# Autodesk Inventor assembly: Assembly
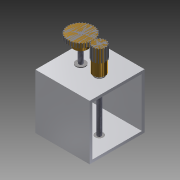
[picture p0: Inventor's stored thumbnail of the model, 180x180]
Saved by Autodesk Inventor 2015 (Build 190159000, 159)
## iProperties
Created: 2015-06-23
Part Number: Assembly
Document SubType Name: Assembly
Designer: kenta
Author: kenta
## Documents named in this file (9)
- C:\Users\kenta\Documents\Inventor\知能ロボコン\Poster presentation\Assembly1.iam
- C:\Users\kenta\Documents\Inventor\知能ロボコン\Poster presentation\Square pipe.ipt
- C:\Users\kenta\Documents\Inventor\知能ロボコン\Poster presentation\Bearing_MF63ZZ.ipt
- C:\Users\kenta\Documents\Inventor\知能ロボコン\Poster presentation\S50B 18K+0803.ipt
- C:\Users\kenta\Documents\Inventor\知能ロボコン\Poster presentation\S50B 36B+0303.ipt
- C:\Users\kenta\Documents\Inventor\知能ロボコン\Poster presentation\Stopper.ipt
- C:\Users\kenta\Documents\Inventor\知能ロボコン\Poster presentation\Shaft 65mm.ipt
- C:\Users\健太\Documents\Inventor\知能ロボコン\Poster presentation\Assembly1\デザイン アクセラレータ\平歯車1.iam
- C:\Users\kenta\Documents\Inventor\知能ロボコン\Poster presentation\Assembly1\デザイン アクセラレータ\平歯車1.iam
## Components (13 placed, 7 different names)
1. Square pipe:1 — 挿入:1, 挿入:2, 挿入:3, 挿入:4, メイト:1
2. Bearing_MF63ZZ:1 — 挿入:1, 挿入:7
3. Bearing_MF63ZZ:2 — 挿入:2, 挿入:8
4. Bearing_MF63ZZ:3 — 挿入:3, 挿入:9
5. Bearing_MF63ZZ:4 — 挿入:4, 挿入:11
6. S50B 18K+0803:1 — 挿入:7, メイト:3, フラッシュ:2, フラッシュ:4
7. S50B 36B+0303:1 — 挿入:8, メイト:2, フラッシュ:1, 挿入:12, メイト:4, フラッシュ:3
8. Stopper:1 — 挿入:11
9. Stopper:2 — 挿入:9, 挿入:10
10. Shaft 65mm:1 — 挿入:10, メイト:5
11. 平歯車:1 [sub-assembly] — メイト:2, フラッシュ:1, メイト:3, フラッシュ:2
12. Shaft 65mm:2 — 挿入:12
13. 平歯車:1 [sub-assembly] — メイト:4, フラッシュ:3, メイト:5, フラッシュ:4
## Relationships (19: Insert 10, Mate 5, Flush 4)
- 挿入:1 [Insert]: Square pipe:1 ↔ Bearing_MF63ZZ:1
- 挿入:2 [Insert]: Square pipe:1 ↔ Bearing_MF63ZZ:2
- 挿入:3 [Insert]: Square pipe:1 ↔ Bearing_MF63ZZ:3
- 挿入:4 [Insert]: Square pipe:1 ↔ Bearing_MF63ZZ:4
- 挿入:7 [Insert] (1 mm): Bearing_MF63ZZ:1 ↔ S50B 18K+0803:1
- 挿入:8 [Insert] (-19 mm): Bearing_MF63ZZ:2 ↔ S50B 36B+0303:1
- 挿入:9 [Insert]: Bearing_MF63ZZ:3 ↔ Stopper:2
- 挿入:10 [Insert]: Stopper:2 ↔ Shaft 65mm:1
- 挿入:11 [Insert]: Bearing_MF63ZZ:4 ↔ Stopper:1
- メイト:1 [Mate]: Square pipe:1
- メイト:2 [Mate]: S50B 36B+0303:1 ↔ 平歯車:1
- フラッシュ:1 [Flush]: S50B 36B+0303:1 ↔ 平歯車:1
- メイト:3 [Mate]: S50B 18K+0803:1 ↔ 平歯車:1
- フラッシュ:2 [Flush]: S50B 18K+0803:1 ↔ 平歯車:1
- 挿入:12 [Insert]: S50B 36B+0303:1 ↔ Shaft 65mm:2
- メイト:4 [Mate]: S50B 36B+0303:1 ↔ 平歯車:1
- フラッシュ:3 [Flush]: S50B 36B+0303:1 ↔ 平歯車:1
- メイト:5 [Mate]: Shaft 65mm:1 ↔ 平歯車:1
- フラッシュ:4 [Flush]: S50B 18K+0803:1 ↔ 平歯車:1
